# Autodesk Inventor assembly: Ensamblaje1
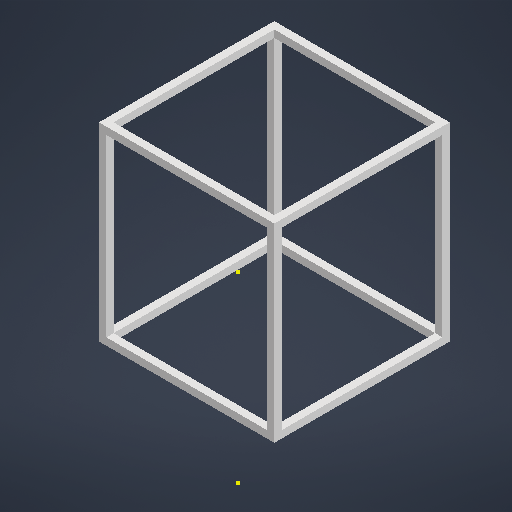
[picture p0: Inventor's stored thumbnail of the model, 512x512]
Saved by Autodesk Inventor 2027 (Build 310192000, 192)
## iProperties
Created: 2026-04-01
Part Number: Ensamblaje1
Document SubType Name: Assembly
Designer: leand
Author: leand
## Documents named in this file (3)
- C:\Users\leand\OneDrive\Desktop\Ensamblaje1.iam
- C:\Users\leand\OneDrive\Desktop\Pieza1.ipt
- C:\Users\leand\OneDrive\Desktop\Pieza2.ipt
## Components (6 placed, 2 different names)
1. Pieza1:1 — Coincidencia:1, Coincidencia:2, Coincidencia:3, Coincidencia:4
2. Pieza1:2 — Coincidencia:5
3. Pieza2:1 — Coincidencia:2, Coincidencia:5
4. Pieza2:2 — Coincidencia:1
5. Pieza2:3 — Coincidencia:3
6. Pieza2:4 — Coincidencia:4
## Relationships (5: Mate 5)
- Coincidencia:1 [Mate]: Pieza1:1 ↔ Pieza2:2
- Coincidencia:2 [Mate]: Pieza1:1 ↔ Pieza2:1
- Coincidencia:3 [Mate]: Pieza1:1 ↔ Pieza2:3
- Coincidencia:4 [Mate]: Pieza1:1 ↔ Pieza2:4
- Coincidencia:5 [Mate]: Pieza1:2 ↔ Pieza2:1
